# Autodesk Inventor assembly: 3136 1149 25
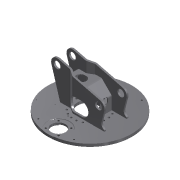
[picture p0: Inventor's stored thumbnail of the model, 180x180]
Saved by Autodesk Inventor 2022 Beta2 (Build 260130000, 130) ContinuousBuild 0
## iProperties
Shininess: 0.0
Length Units: 11269
Angle Units: 11279
Time Units: 11290
Mass Units: 11283
Length Display Precision: 3
Angle Display Precision: 2
Created: 2000-09-12
Part Number: 3136 1149 25
Description: Armbracket
Document SubType Name: Assembly
Designer: Joe M
Engineer: Joe M
Density: 7.860000000000001
Volumn: 3631.4488536095237
Area: 6993.527199222248
PropertySet Name: Model Information
Control State: 0
Master: False
Checked Out: False
Last Check In By: Administratör
Last Check In Date: 2002-03-08
Title: Arminfästning svängmotor
Author: Joe M
## Documents named in this file (5)
- C:\Autodesk Inventor 2021 Intro Practice Files\BOM\3136 1149 25.iam
- C:\Autodesk Inventor 2021 Intro Practice Files\BOM\3136 1149 26.ipt
- C:\Autodesk Inventor 2021 Intro Practice Files\BOM\3136 1149 28.ipt
- C:\Autodesk Inventor 2021 Intro Practice Files\BOM\3136 1149 27.ipt
- C:\Autodesk Inventor 2021 Intro Practice Files\BOM\3136 1149 29.ipt
## Components (4 placed, 4 different names)
1. 3136 1149 26:1 — Mate:1, Mate:2, Mate:3, Mate:4, Mate:5, Mate:9, Mate:10, Mate:11, Mate:12
2. 3136 1149 28:1 — Mate:1, Mate:3, Mate:11
3. 3136 1149 27:1 — Mate:4, Mate:5, Mate:10
4. 3136 1149 29:1 — Mate:2, Mate:9, Mate:12
## Relationships (9: Mate 9)
- Mate:1: 3136 1149 26:1 ↔ 3136 1149 28:1
- Mate:2: 3136 1149 26:1 ↔ 3136 1149 29:1
- Mate:3: 3136 1149 26:1 ↔ 3136 1149 28:1
- Mate:4: 3136 1149 26:1 ↔ 3136 1149 27:1
- Mate:5: 3136 1149 26:1 ↔ 3136 1149 27:1
- Mate:9: 3136 1149 26:1 ↔ 3136 1149 29:1
- Mate:10 (0.15 mm): 3136 1149 26:1 ↔ 3136 1149 27:1
- Mate:11 (0.15 mm): 3136 1149 26:1 ↔ 3136 1149 28:1
- Mate:12 (0.15 mm): 3136 1149 26:1 ↔ 3136 1149 29:1
